# Autodesk Inventor assembly: МПСТ Редуктор
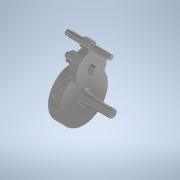
[picture p0: Inventor's stored thumbnail of the model, 180x180]
Saved by Autodesk Inventor 2022 (Build 260153070, 153G)
## iProperties
Created: 2021-09-16
Part Number: МПСТ Редуктор
Document SubType Name: Assembly
Designer: Алексанян Г.
Author: Алексанян Г.
## Documents named in this file (12)
- C:\Users\Гарник\Desktop\учёба\5 семак\Детмаш\Reductor\МПСТ Редуктор.iam
- C:\Users\Гарник\Desktop\учёба\5 семак\Детмаш\Reductor\МПСТ Промежуточный Вал.iam
- C:\Users\Гарник\Desktop\учёба\5 семак\Детмаш\Reductor\МПСТ Тихоходный Вал.iam
- C:\Users\Гарник\Desktop\учёба\5 семак\Детмаш\Reductor\МПСТ Быстроходный Вал.iam
- C:\Users\Гарник\Desktop\учёба\5 семак\Детмаш\Reductor\МПСТ Редуктор\Мастер проектирования\Цилиндрическое зубчатое зацепление11.ipt
- C:\Users\Гарник\Desktop\учёба\5 семак\Детмаш\Reductor\МПСТ Редуктор\Мастер проектирования\Цилиндрическое зубчатое зацепление21.ipt
- C:\Users\Гарник\Desktop\учёба\5 семак\Детмаш\Reductor\МПСТ Шпонка тихоходного вала.ipt
- C:\Users\Гарник\Desktop\учёба\5 семак\Детмаш\Reductor\МПСТ Шпонка переходного вала.ipt
- C:\Users\Гарник\Desktop\учёба\5 семак\Детмаш\Reductor\МПСТ Редуктор\Мастер проектирования\Цилиндрическое зубчатое зацепление12.ipt
- C:\Users\Гарник\Desktop\учёба\5 семак\Детмаш\Reductor\МПСТ Редуктор\Мастер проектирования\Цилиндрическое зубчатое зацепление22.ipt
- C:\Users\Гарник\Documents\Inventor\Content Center Files\R2022\ru-RU\Bearing 116000 GOST 8995-75\Подшипник 116117 ГОСТ 8995-75.ipt
- C:\Users\Гарник\Documents\Inventor\Content Center Files\R2022\ru-RU\Bearing 116000 GOST 8995-75\Подшипник 116120 ГОСТ 8995-75.ipt
## Components (11 placed, 9 different names)
1. МПСТ Промежуточный Вал:1 [sub-assembly] — Совмещение:1, Совмещение:5, Заподлицо:5, Совмещение:19, Вставка:3, ЗубчПер:2, Вставка:4, Вставка:5, Совмещение:25
2. МПСТ Тихоходный Вал:1 [sub-assembly] — Совмещение:1, Заподлицо:5, Заподлицо:6, Совмещение:16, Совмещение:18, Совмещение:21, Совмещение:22, Вставка:1, Совмещение:24, Совмещение:28, Совмещение:30
3. МПСТ Быстроходный Вал:1 [sub-assembly] — Совмещение:5, Заподлицо:6, Совмещение:20, Вставка:6, ЗубчПер:4
4. Цилиндрическое зубчатое зацепление1:1 — Вставка:3, ЗубчПер:1, ЗубчПер:2, Совмещение:27
5. Цилиндрическое зубчатое зацепление2:1 — Совмещение:22, Совмещение:23, Совмещение:24, ЗубчПер:1, Совмещение:29, Совмещение:31
6. МПСТ Шпонка тихоходного вала:1 — Вставка:1, Совмещение:23
7. МПСТ Шпонка переходного вала:1 — Вставка:4, Вставка:5, Совмещение:26
8. Цилиндрическое зубчатое зацепление1:2 — Вставка:6, ЗубчПер:3, ЗубчПер:4
9. Цилиндрическое зубчатое зацепление2:2 — Совмещение:25, Совмещение:26, Совмещение:27, ЗубчПер:3
10. Подшипник 116000 ГОСТ 8995-75 116117:1 — Совмещение:28, Совмещение:29
11. Подшипник 116000 ГОСТ 8995-75 116120:1 — Совмещение:30, Совмещение:31
## Relationships (28: Mate 17, Insert 5, RelateRotation 4, Flush 2)
- Совмещение:1 [Mate] (300 mm): МПСТ Промежуточный Вал:1 ↔ МПСТ Тихоходный Вал:1
- Совмещение:5 [Mate] (200 mm): МПСТ Промежуточный Вал:1 ↔ МПСТ Быстроходный Вал:1
- Заподлицо:5 [Flush]: МПСТ Промежуточный Вал:1 ↔ МПСТ Тихоходный Вал:1
- Заподлицо:6 [Flush]: МПСТ Тихоходный Вал:1 ↔ МПСТ Быстроходный Вал:1
- Совмещение:16 [Mate]: МПСТ Тихоходный Вал:1
- Совмещение:18 [Mate]: МПСТ Тихоходный Вал:1
- Совмещение:19 [Mate]: МПСТ Промежуточный Вал:1
- Совмещение:20 [Mate]: МПСТ Быстроходный Вал:1
- Совмещение:21 [Mate]: МПСТ Тихоходный Вал:1
- Совмещение:22 [Mate]: МПСТ Тихоходный Вал:1 ↔ Цилиндрическое зубчатое зацепление2:1
- Вставка:1 [Insert]: МПСТ Тихоходный Вал:1 ↔ МПСТ Шпонка тихоходного вала:1
- Совмещение:23 [Mate]: Цилиндрическое зубчатое зацепление2:1 ↔ МПСТ Шпонка тихоходного вала:1
- Совмещение:24 [Mate]: МПСТ Тихоходный Вал:1 ↔ Цилиндрическое зубчатое зацепление2:1
- Вставка:3 [Insert]: МПСТ Промежуточный Вал:1 ↔ Цилиндрическое зубчатое зацепление1:1
- ЗубчПер:1 [RelateRotation] (5.0789 ul): Цилиндрическое зубчатое зацепление1:1 ↔ Цилиндрическое зубчатое зацепление2:1
- ЗубчПер:2 [RelateRotation] (1 ul): МПСТ Промежуточный Вал:1 ↔ Цилиндрическое зубчатое зацепление1:1
- Вставка:4 [Insert]: МПСТ Промежуточный Вал:1 ↔ МПСТ Шпонка переходного вала:1
- Вставка:5 [Insert]: МПСТ Промежуточный Вал:1 ↔ МПСТ Шпонка переходного вала:1
- Совмещение:25 [Mate]: МПСТ Промежуточный Вал:1 ↔ Цилиндрическое зубчатое зацепление2:2
- Совмещение:26 [Mate]: МПСТ Шпонка переходного вала:1 ↔ Цилиндрическое зубчатое зацепление2:2
- Совмещение:27 [Mate]: Цилиндрическое зубчатое зацепление1:1 ↔ Цилиндрическое зубчатое зацепление2:2
- Вставка:6 [Insert]: МПСТ Быстроходный Вал:1 ↔ Цилиндрическое зубчатое зацепление1:2
- ЗубчПер:3 [RelateRotation] (3.825 ul): Цилиндрическое зубчатое зацепление1:2 ↔ Цилиндрическое зубчатое зацепление2:2
- ЗубчПер:4 [RelateRotation] (1 ul): МПСТ Быстроходный Вал:1 ↔ Цилиндрическое зубчатое зацепление1:2
- Совмещение:28 [Mate]: МПСТ Тихоходный Вал:1 ↔ Подшипник 116000 ГОСТ 8995-75 116117:1
- Совмещение:29 [Mate]: Цилиндрическое зубчатое зацепление2:1 ↔ Подшипник 116000 ГОСТ 8995-75 116117:1
- Совмещение:30 [Mate]: МПСТ Тихоходный Вал:1 ↔ Подшипник 116000 ГОСТ 8995-75 116120:1
- Совмещение:31 [Mate]: Цилиндрическое зубчатое зацепление2:1 ↔ Подшипник 116000 ГОСТ 8995-75 116120:1
